# Autodesk Inventor assembly: Prototype_03
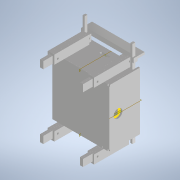
[picture p0: Inventor's stored thumbnail of the model, 180x180]
Saved by Autodesk Inventor 2020 (Build 240168000, 168)
## iProperties
Created: 2019-12-19
Part Number: Prototype_03
Document SubType Name: Assembly
Designer: damien
Author: damien
## Documents named in this file (3)
- D:\fablab\save\Prototype_03.iam
- D:\fablab\save\BOX_PART.iam
- D:\fablab\save\Foot.iam
## Components (5 placed, 2 different names)
1. BOX_PART:1 [sub-assembly] — Placage:1, Placage:2, Placage:3, Placage:4, Placage:5, Placage:6, Placage:7, Placage:8, Placage:9
2. Foot:1 [sub-assembly] — Placage:4, Placage:5, Placage:6
3. Foot:2 [sub-assembly] — Placage:1, Placage:2, Placage:3
4. Foot:3 [sub-assembly]
5. Foot:4 [sub-assembly] — Placage:7, Placage:8, Placage:9
## Relationships (9: Mate 9)
- Placage:1 [Mate]: BOX_PART:1 ↔ Foot:2
- Placage:2 [Mate]: BOX_PART:1 ↔ Foot:2
- Placage:3 [Mate]: BOX_PART:1 ↔ Foot:2
- Placage:4 [Mate]: BOX_PART:1 ↔ Foot:1
- Placage:5 [Mate]: BOX_PART:1 ↔ Foot:1
- Placage:6 [Mate]: BOX_PART:1 ↔ Foot:1
- Placage:7 [Mate]: BOX_PART:1 ↔ Foot:4
- Placage:8 [Mate]: BOX_PART:1 ↔ Foot:4
- Placage:9 [Mate]: BOX_PART:1 ↔ Foot:4
